# Autodesk Inventor assembly: BBM Staging Plate Assembly
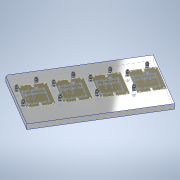
[picture p0: Inventor's stored thumbnail of the model, 180x180]
Saved by Autodesk Inventor 2022 (Build 260153000, 153)
## iProperties
Created: 2021-01-11
Part Number: BBM Staging Plate Assembly
Document SubType Name: Assembly
Designer: caleb
Author: caleb
## Documents named in this file (4)
- C:\Users\Caleb\Desktop\nebraska-silicon-lab\Hardware\ETL\Module Assembly\Baseplate Staging Plate - V1\Baseplate Staging Plate Assembly - V1.iam
- C:\Users\Caleb\Desktop\nebraska-silicon-lab\Hardware\ETL\Module Assembly\Baseplate Staging Plate - V1\Baseplate Staging Plate - V1.ipt
- C:\Users\Caleb\Desktop\nebraska-silicon-lab\Hardware\ETL\Module Assembly\Baseplate Staging Plate - V1\8472A51_Locating Pin.ipt
- C:\Users\Caleb\Desktop\nebraska-silicon-lab\Hardware\ETL\modules\etl standard baseplate with cutouts.ipt
## Components (17 placed, 3 different names)
1. Baseplate Staging Plate - V1:1 — Insert:1, Insert:2, Insert:3, Mate:1, Insert:4, Insert:5, Insert:6, Mate:2, Insert:7, Insert:8, Insert:9, Insert:10, Insert:11, Insert:12, Mate:3, Mate:4
2. 8472A51_Locating Pin:1 — Insert:1, Tangent:2
3. 8472A51_Locating Pin:2 — Insert:2, Tangent:1
4. 8472A51_Locating Pin:3 — Insert:3, Tangent:3
5. etl standard baseplate with cutouts:1 — Mate:1, Tangent:1, Tangent:2, Tangent:3
6. 8472A51_Locating Pin:4 — Insert:5
7. 8472A51_Locating Pin:5 — Insert:6
8. 8472A51_Locating Pin:6 — Insert:4
9. etl standard baseplate with cutouts:2 — Mate:2
10. 8472A51_Locating Pin:7 — Insert:8
11. 8472A51_Locating Pin:8 — Insert:9
12. 8472A51_Locating Pin:9 — Insert:7
13. etl standard baseplate with cutouts:3 — Mate:3
14. 8472A51_Locating Pin:10 — Insert:11
15. 8472A51_Locating Pin:11 — Insert:12
16. 8472A51_Locating Pin:12 — Insert:10
17. etl standard baseplate with cutouts:4 — Mate:4
## Relationships (28: Insert 12, Tangent 12, Mate 4)
- Insert:1: Baseplate Staging Plate - V1:1 ↔ 8472A51_Locating Pin:1
- Insert:2: Baseplate Staging Plate - V1:1 ↔ 8472A51_Locating Pin:2
- Insert:3: Baseplate Staging Plate - V1:1 ↔ 8472A51_Locating Pin:3
- Mate:1: Baseplate Staging Plate - V1:1 ↔ etl standard baseplate with cutouts:1
- Tangent:1: 8472A51_Locating Pin:2 ↔ etl standard baseplate with cutouts:1
- Tangent:2: 8472A51_Locating Pin:1 ↔ etl standard baseplate with cutouts:1
- Tangent:3: 8472A51_Locating Pin:3 ↔ etl standard baseplate with cutouts:1
- [Tangent]: 8472A51_Locating Pin:5 ↔ etl standard baseplate with cutouts:2
- [Tangent]: 8472A51_Locating Pin:4 ↔ etl standard baseplate with cutouts:2
- [Tangent]: 8472A51_Locating Pin:6 ↔ etl standard baseplate with cutouts:2
- [Tangent]: 8472A51_Locating Pin:8 ↔ etl standard baseplate with cutouts:3
- [Tangent]: 8472A51_Locating Pin:7 ↔ etl standard baseplate with cutouts:3
- [Tangent]: 8472A51_Locating Pin:9 ↔ etl standard baseplate with cutouts:3
- [Tangent]: 8472A51_Locating Pin:11 ↔ etl standard baseplate with cutouts:4
- [Tangent]: 8472A51_Locating Pin:10 ↔ etl standard baseplate with cutouts:4
- [Tangent]: 8472A51_Locating Pin:12 ↔ etl standard baseplate with cutouts:4
- Insert:4: Baseplate Staging Plate - V1:1 ↔ 8472A51_Locating Pin:6
- Insert:5: Baseplate Staging Plate - V1:1 ↔ 8472A51_Locating Pin:4
- Insert:6: Baseplate Staging Plate - V1:1 ↔ 8472A51_Locating Pin:5
- Mate:2: Baseplate Staging Plate - V1:1 ↔ etl standard baseplate with cutouts:2
- Insert:7: Baseplate Staging Plate - V1:1 ↔ 8472A51_Locating Pin:9
- Insert:8: Baseplate Staging Plate - V1:1 ↔ 8472A51_Locating Pin:7
- Insert:9: Baseplate Staging Plate - V1:1 ↔ 8472A51_Locating Pin:8
- Insert:10: Baseplate Staging Plate - V1:1 ↔ 8472A51_Locating Pin:12
- Insert:11: Baseplate Staging Plate - V1:1 ↔ 8472A51_Locating Pin:10
- Insert:12: Baseplate Staging Plate - V1:1 ↔ 8472A51_Locating Pin:11
- Mate:3: Baseplate Staging Plate - V1:1 ↔ etl standard baseplate with cutouts:3
- Mate:4: Baseplate Staging Plate - V1:1 ↔ etl standard baseplate with cutouts:4
## Named parameters: d66_d50 = 0 mm, d67_d48 = 0 mm, d68_d49 = 0 mm, d69_d50 = 0 mm, d70_d48 = 0 mm, d71_d49 = 0 mm, d72_d50 = 0 mm, d73_d48 = 0 mm, d74_d49 = 0 mm
